# Autodesk Inventor assembly: Assembly
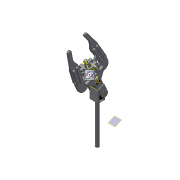
[picture p0: Inventor's stored thumbnail of the model, 180x180]
Saved by Autodesk Inventor 2018 (Build 220112000, 112)
## iProperties
Created: 2018-02-18
Part Number: Assembly
Document SubType Name: Assembly
Designer: Bardo91
Author: Bardo91
## Documents named in this file (10)
- E:\programming\hecatonquiros\cad_models\tools\gripper\serial_model_5DoF\Assembly.iam
- E:\programming\hecatonquiros\cad_models\tools\gripper\serial_model_5DoF\core_structure.ipt
- E:\programming\hecatonquiros\cad_models\tools\gripper\serial_model_5DoF\microservo_FT.ipt
- E:\programming\hecatonquiros\cad_models\tools\gripper\serial_model_5DoF\base_gripper.ipt
- E:\programming\hecatonquiros\cad_models\tools\gripper\serial_model_5DoF\bar.ipt
- E:\programming\hecatonquiros\cad_models\tools\gripper\serial_model_5DoF\barMini.ipt
- E:\programming\hecatonquiros\cad_models\tools\gripper\serial_model_5DoF\holdBar.ipt
- E:\programming\hecatonquiros\cad_models\tools\gripper\serial_model_5DoF\gripper.ipt
- E:\programming\hecatonquiros\cad_models\tools\gripper\serial_model_5DoF\ScrewActuatorGripper.ipt
- E:\programming\hecatonquiros\cad_models\tools\gripper\serial_model_5DoF\ScrewActuatorGripperCenter.ipt
## Components (20 placed, 9 different names)
1. core_structure:1 — Mate:1, Mate:2, Mate:3
2. microservo_FT:1 — Mate:1, Mate:2, Mate:3, Mate:4, Flush:1
3. base_gripper:1 — Mate:4, Flush:1, Mate:5, Mate:6, Mate:7, Mate:8, Mate:9, Mate:10, Mate:11, Mate:12, Mate:13
4. microservo_FT:2 — Mate:5, Mate:6, Mate:7, Mate:40, Mate:41
5. bar:1 — Mate:27, Mate:28, Mate:39, Mate:44, Mate:47
6. bar:2 — Mate:29, Mate:30, Mate:38
7. bar:3 — Mate:31, Mate:34, Mate:36
8. bar:4 — Mate:32, Mate:33, Mate:35, Mate:37
9. bar:5 — Mate:14, Mate:15, Mate:22
10. bar:6 — Mate:16, Mate:17, Mate:24
11. bar:7 — Mate:18, Mate:19, Mate:26
12. bar:8 — Mate:20, Mate:21, Mate:23, Mate:25, Mate:43, Mate:46
13. barMini:1 — Mate:44, Mate:47, Mate:48
14. barMini:2 — Mate:43, Mate:45, Mate:46
15. holdBar:1 — Mate:11, Mate:12, Mate:13, Mate:14, Mate:15, Mate:16, Mate:17, Mate:18, Mate:19, Mate:20, Mate:21
16. holdBar:2 — Mate:8, Mate:9, Mate:10, Mate:27, Mate:28, Mate:29, Mate:30, Mate:31, Mate:32, Mate:33, Mate:34
17. gripper:1 — Mate:22, Mate:23, Mate:24, Mate:25, Mate:26
18. gripper:2 — Mate:35, Mate:36, Mate:37, Mate:38, Mate:39
19. ScrewActuatorGripper:1 — Mate:40, Mate:41, Mate:42
20. ScrewActuatorGripperCenter:1 — Mate:42, Mate:45, Mate:48
## Relationships (49: Mate 48, Flush 1)
- Mate:1: core_structure:1 ↔ microservo_FT:1
- Mate:2: core_structure:1 ↔ microservo_FT:1
- Mate:3: core_structure:1 ↔ microservo_FT:1
- Mate:4: microservo_FT:1 ↔ base_gripper:1
- Flush:1: microservo_FT:1 ↔ base_gripper:1
- Mate:5: base_gripper:1 ↔ microservo_FT:2
- Mate:6: base_gripper:1 ↔ microservo_FT:2
- Mate:7: base_gripper:1 ↔ microservo_FT:2
- Mate:8: base_gripper:1 ↔ holdBar:2
- Mate:9: base_gripper:1 ↔ holdBar:2
- Mate:10: base_gripper:1 ↔ holdBar:2
- Mate:11: base_gripper:1 ↔ holdBar:1
- Mate:12: base_gripper:1 ↔ holdBar:1
- Mate:13: base_gripper:1 ↔ holdBar:1
- Mate:14: bar:5 ↔ holdBar:1
- Mate:15: bar:5 ↔ holdBar:1
- Mate:16: bar:6 ↔ holdBar:1
- Mate:17: bar:6 ↔ holdBar:1
- Mate:18: bar:7 ↔ holdBar:1
- Mate:19: bar:7 ↔ holdBar:1
- Mate:20: bar:8 ↔ holdBar:1
- Mate:21: bar:8 ↔ holdBar:1
- Mate:22: bar:5 ↔ gripper:1
- Mate:23: bar:8 ↔ gripper:1
- Mate:24: bar:6 ↔ gripper:1
- Mate:25: bar:8 ↔ gripper:1
- Mate:26: bar:7 ↔ gripper:1
- Mate:27: bar:1 ↔ holdBar:2
- Mate:28: bar:1 ↔ holdBar:2
- Mate:29: bar:2 ↔ holdBar:2
- Mate:30: bar:2 ↔ holdBar:2
- Mate:31: bar:3 ↔ holdBar:2
- Mate:32: bar:4 ↔ holdBar:2
- Mate:33: bar:4 ↔ holdBar:2
- Mate:34: bar:3 ↔ holdBar:2
- Mate:35: bar:4 ↔ gripper:2
- Mate:36: bar:3 ↔ gripper:2
- Mate:37: bar:4 ↔ gripper:2
- Mate:38: bar:2 ↔ gripper:2
- Mate:39: bar:1 ↔ gripper:2
- Mate:40: microservo_FT:2 ↔ ScrewActuatorGripper:1
- Mate:41: microservo_FT:2 ↔ ScrewActuatorGripper:1
- Mate:42: ScrewActuatorGripper:1 ↔ ScrewActuatorGripperCenter:1
- Mate:43: bar:8 ↔ barMini:2
- Mate:44: bar:1 ↔ barMini:1
- Mate:45: barMini:2 ↔ ScrewActuatorGripperCenter:1
- Mate:46: bar:8 ↔ barMini:2
- Mate:47: bar:1 ↔ barMini:1
- Mate:48: barMini:1 ↔ ScrewActuatorGripperCenter:1
